# Autodesk Inventor assembly: Correct nut unmodified ASSembly
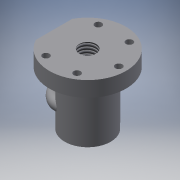
[picture p0: Inventor's stored thumbnail of the model, 180x180]
Saved by Autodesk Inventor 2016 (Build 200138000, 138)
## iProperties
Created: 2017-07-25
Part Number: Correct nut unmodified ASSembly
Document SubType Name: Assembly
Designer: M227562
Author: M227562
## Documents named in this file (3)
- C:\Users\M227562\Desktop\Correct nut unmodified ASSembly.iam
- C:\Users\M227562\Documents\Tube for ball screew.ipt
- C:\Users\M227562\Desktop\NUT TEST.ipt
## Components (2 placed, 2 different names)
1. Tube for ball screew:1 — Rotational:1
2. NUT TEST:1 — Rotational:1
## Relationships (1: RevoluteJoint 1)
- Rotational:1 [RevoluteJoint] (-1.8 mm): Tube for ball screew:1 ↔ NUT TEST:1
